# Autodesk Inventor assembly: EL2-GB-100
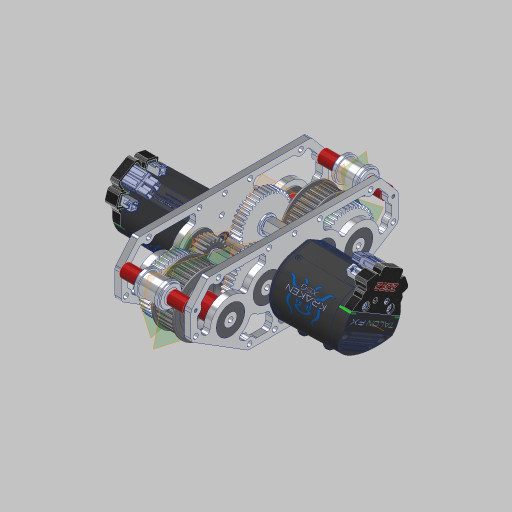
[picture p0: Inventor's stored thumbnail of the model, 512x512]
Saved by Autodesk Inventor 2023.5 (Build 275446000, 446)
## iProperties
Created: 2025-01-18
Part Number: EL2-GB-100
Document SubType Name: Assembly
Designer: jmcintyr
Author: jmcintyr
## Documents named in this file (17)
- C:\Users\slick\OneDrive\Desktop\2025-ReefScape---CAD\Elevator\EL2-GB\EL2-GB-100.iam
- C:\Users\slick\OneDrive\Desktop\2025-ReefScape---CAD\Elevator\EL2-GB\EL2-GB-001.ipt
- C:\Users\slick\OneDrive\Desktop\2025-ReefScape---CAD\Elevator\EL2-GB\EL2-GB-002.ipt
- C:\Users\slick\OneDrive\Desktop\2025-ReefScape---CAD\COMMON PARTS\MOTORS\Kracken with Cover and Boards.iam
- C:\Users\slick\OneDrive\Desktop\2025-ReefScape---CAD\COMMON PARTS\BEARINGS\0_500_ID_x_1_125_OD_x_0_313_WD_Flanged_Bearing_217-2731.ipt
- C:\Users\slick\OneDrive\Desktop\2025-ReefScape---CAD\COMMON PARTS\GEARS\20dp .5 hex\20t_Aluminum_Spur_Gear_20_DP_1_2_Hex_Bore_217-2702.ipt
- C:\Users\slick\OneDrive\Desktop\2025-ReefScape---CAD\COMMON PARTS\GEARS\20dp .5 hex\40t_Aluminum_Spur_Gear_20_DP_1_2_Hex_Bore_217-2708.ipt
- C:\Users\slick\OneDrive\Desktop\2025-ReefScape---CAD\COMMON PARTS\PULLEYS\htd\36t_x_15mm_Wide_Aluminum_Pulley_HTD_5mm_1_2_Hex_217-4103.ipt
- C:\Users\slick\OneDrive\Desktop\2025-ReefScape---CAD\Elevator\EL2-GB\EL2-GB-200.iam
- C:\Users\slick\OneDrive\Desktop\2025-ReefScape---CAD\Elevator\EL2-GB\EL2-GB-003.ipt
- C:\Users\slick\OneDrive\Desktop\2025-ReefScape---CAD\Elevator\EL2-GB\EL2-GB-004Spacer.ipt
- C:\Users\slick\OneDrive\Desktop\2025-ReefScape---CAD\Elevator\EL2-GB\EL2-GB-005E-grove.ipt
- C:\Users\slick\OneDrive\Desktop\2025-ReefScape---CAD\Elevator\EL2-GB\EL2-GB-006Spacer.ipt
- C:\Users\slick\OneDrive\Desktop\2025-ReefScape---CAD\Elevator\EL2-GB\EL2-GB-007Spacer.ipt
- C:\Users\slick\OneDrive\Desktop\2025-ReefScape---CAD\Elevator\EL2-GB\EL2-GB-008.ipt
- C:\Users\slick\OneDrive\Desktop\2025-ReefScape---CAD\Elevator\EL2-GB\EL2-GB-009Spacer.ipt
- C:\Users\slick\OneDrive\Desktop\2025-ReefScape---CAD\COMMON PARTS\GEARS\WCP-1006\WCP-1006.ipt
## Components (46 placed, 16 different names)
1. EL2-GB-001:1 — Insert:3, Insert:4, Insert:10, Insert:11, Insert:16, Insert:17, Insert:18, Insert:19, Symmetry:1, Mate:18, Mate:45, Insert:27, Mate:49
2. EL2-GB-001:2 — Insert:8, Insert:9, Insert:12, Insert:13, Insert:14, Insert:15, Symmetry:1, Insert:24, Insert:25, Insert:26, Mate:46, Mate:50
3. EL2-GB-002:1 — Insert:3, Insert:25
4. EL2-GB-002:5 — Insert:4, Insert:24
5. Kracken with Cover and Boards:1 [sub-assembly] — Insert:8, Insert:9
6. Kracken with Cover and Boards:2 [sub-assembly] — Insert:10, Insert:11
7. 0_500_ID_x_1_125_OD_x_0_313_WD_Flanged_Bearing_217-2731:1 — Insert:16, Mate:7, Insert:20, Mate:39, Mate:40
8. 0_500_ID_x_1_125_OD_x_0_313_WD_Flanged_Bearing_217-2731:2 — Insert:17, Insert:21, Mate:33, Mate:34, Mate:35
9. 0_500_ID_x_1_125_OD_x_0_313_WD_Flanged_Bearing_217-2731:3 — Insert:18, Mate:14
10. 0_500_ID_x_1_125_OD_x_0_313_WD_Flanged_Bearing_217-2731:4 — Insert:19, Mate:13, Insert:22, Mate:25, Mate:27
11. 0_500_ID_x_1_125_OD_x_0_313_WD_Flanged_Bearing_217-2731:5 — Insert:12, Mate:10, Mate:37, Mate:38, Mate:42
12. 0_500_ID_x_1_125_OD_x_0_313_WD_Flanged_Bearing_217-2731:6 — Insert:13, Mate:5, Mate:6, Mate:36
13. 0_500_ID_x_1_125_OD_x_0_313_WD_Flanged_Bearing_217-2731:7 — Insert:14, Mate:11, Insert:23, Mate:29, Mate:30, Mate:31
14. 0_500_ID_x_1_125_OD_x_0_313_WD_Flanged_Bearing_217-2731:8 — Insert:15, Mate:23
15. 20t_Aluminum_Spur_Gear_20_DP_1_2_Hex_Bore_217-2702:1 — Mate:6, Mate:22, Flush:4
16. 20t_Aluminum_Spur_Gear_20_DP_1_2_Hex_Bore_217-2702:2 — Mate:14, Mate:20, Flush:6, Mate:32
17. WCP-1006:1
18. WCP-1006:2
19. 40t_Aluminum_Spur_Gear_20_DP_1_2_Hex_Bore_217-2708:1 — Mate:11, Flush:5
20. 40t_Aluminum_Spur_Gear_20_DP_1_2_Hex_Bore_217-2708:2 — Mate:5
21. 40t_Aluminum_Spur_Gear_20_DP_1_2_Hex_Bore_217-2708:3 — Mate:7, Mate:22, Mate:41
22. 36t_x_15mm_Wide_Aluminum_Pulley_HTD_5mm_1_2_Hex_217-4103:1 — Mate:9, Mate:10, Mate:15
23. 40t_Aluminum_Spur_Gear_20_DP_1_2_Hex_Bore_217-2708:4 — Mate:13, Mate:16, Mate:20, Mate:28
24. 36t_x_15mm_Wide_Aluminum_Pulley_HTD_5mm_1_2_Hex_217-4103:2 — Mate:15, Mate:16, Mate:17, Mate:24, Mate:26
25. EL2-GB-200:1 [sub-assembly] — Mate:17, Mate:18
26. EL2-GB-005E-grove:2 — Insert:23, Flush:5, Flush:6
27. EL2-GB-003:2 — Insert:22
28. EL2-GB-005E-grove:1 — Insert:21, Flush:4
29. EL2-GB-003:4 — Insert:20
30. EL2-GB-004Spacer:1 — Mate:23, Mate:24
31. EL2-GB-006Spacer:1 — Mate:25, Mate:26
32. EL2-GB-007Spacer:1 — Mate:27, Mate:28
33. EL2-GB-007Spacer:2 — Mate:29, Mate:30
34. EL2-GB-007Spacer:3 — Mate:31, Mate:32
35. EL2-GB-007Spacer:4 — Mate:33, Mate:36
36. EL2-GB-007Spacer:5 — Mate:34, Mate:35
37. EL2-GB-007Spacer:6 — Mate:37, Mate:42
38. EL2-GB-006Spacer:2 — Mate:38, Mate:41
39. EL2-GB-004Spacer:2 — Mate:39, Mate:40
40. EL2-GB-008:1 — Insert:26, Mate:43, Mate:44
41. EL2-GB-009Spacer:1 — Mate:44, Mate:45
42. EL2-GB-009Spacer:2 — Mate:43, Mate:46
43. EL2-GB-200:2 [sub-assembly] — Flush:7, Mate:51
44. EL2-GB-008:2 — Insert:27, Mate:51
45. EL2-GB-009Spacer:3 — Mate:49
46. EL2-GB-009Spacer:4 — Mate:50
## Relationships (75: Mate 47, Insert 22, Flush 5, Symmetry 1)
- Insert:3: EL2-GB-001:1 ↔ EL2-GB-002:1
- Insert:4: EL2-GB-001:1 ↔ EL2-GB-002:5
- Insert:8: EL2-GB-001:2 ↔ Kracken with Cover and Boards:1
- Insert:9: EL2-GB-001:2 ↔ Kracken with Cover and Boards:1
- Insert:10: EL2-GB-001:1 ↔ Kracken with Cover and Boards:2
- Insert:11: EL2-GB-001:1 ↔ Kracken with Cover and Boards:2
- Insert:12: EL2-GB-001:2 ↔ 0_500_ID_x_1_125_OD_x_0_313_WD_Flanged_Bearing_217-2731:5
- Insert:13: EL2-GB-001:2 ↔ 0_500_ID_x_1_125_OD_x_0_313_WD_Flanged_Bearing_217-2731:6
- Insert:14: EL2-GB-001:2 ↔ 0_500_ID_x_1_125_OD_x_0_313_WD_Flanged_Bearing_217-2731:7
- Insert:15: EL2-GB-001:2 ↔ 0_500_ID_x_1_125_OD_x_0_313_WD_Flanged_Bearing_217-2731:8
- Insert:16: EL2-GB-001:1 ↔ 0_500_ID_x_1_125_OD_x_0_313_WD_Flanged_Bearing_217-2731:1
- Insert:17: EL2-GB-001:1 ↔ 0_500_ID_x_1_125_OD_x_0_313_WD_Flanged_Bearing_217-2731:2
- Insert:18: EL2-GB-001:1 ↔ 0_500_ID_x_1_125_OD_x_0_313_WD_Flanged_Bearing_217-2731:3
- Insert:19: EL2-GB-001:1 ↔ 0_500_ID_x_1_125_OD_x_0_313_WD_Flanged_Bearing_217-2731:4
- [Mate]: Kracken with Cover and Boards:1 ↔ WCP-1006:1
- [Mate]: Kracken with Cover and Boards:2 ↔ WCP-1006:2
- [Mate] (3.175 mm): EL2-GB-001:2 ↔ WCP-1006:1
- [Mate] (3.175 mm): EL2-GB-001:1 ↔ WCP-1006:2
- Mate:5: 0_500_ID_x_1_125_OD_x_0_313_WD_Flanged_Bearing_217-2731:6 ↔ 40t_Aluminum_Spur_Gear_20_DP_1_2_Hex_Bore_217-2708:2
- Mate:6: 0_500_ID_x_1_125_OD_x_0_313_WD_Flanged_Bearing_217-2731:6 ↔ 20t_Aluminum_Spur_Gear_20_DP_1_2_Hex_Bore_217-2702:1
- Mate:7: 0_500_ID_x_1_125_OD_x_0_313_WD_Flanged_Bearing_217-2731:1 ↔ 40t_Aluminum_Spur_Gear_20_DP_1_2_Hex_Bore_217-2708:3
- [Flush]: WCP-1006:2 ↔ 40t_Aluminum_Spur_Gear_20_DP_1_2_Hex_Bore_217-2708:2
- Symmetry:1: EL2-GB-001:1 ↔ EL2-GB-001:2
- Mate:9: 36t_x_15mm_Wide_Aluminum_Pulley_HTD_5mm_1_2_Hex_217-4103:1
- Mate:10: 0_500_ID_x_1_125_OD_x_0_313_WD_Flanged_Bearing_217-2731:5 ↔ 36t_x_15mm_Wide_Aluminum_Pulley_HTD_5mm_1_2_Hex_217-4103:1
- Mate:11: 0_500_ID_x_1_125_OD_x_0_313_WD_Flanged_Bearing_217-2731:7 ↔ 40t_Aluminum_Spur_Gear_20_DP_1_2_Hex_Bore_217-2708:1
- Mate:13: 0_500_ID_x_1_125_OD_x_0_313_WD_Flanged_Bearing_217-2731:4 ↔ 40t_Aluminum_Spur_Gear_20_DP_1_2_Hex_Bore_217-2708:4
- Mate:14: 0_500_ID_x_1_125_OD_x_0_313_WD_Flanged_Bearing_217-2731:3 ↔ 20t_Aluminum_Spur_Gear_20_DP_1_2_Hex_Bore_217-2702:2
- Mate:15: 36t_x_15mm_Wide_Aluminum_Pulley_HTD_5mm_1_2_Hex_217-4103:1 ↔ 36t_x_15mm_Wide_Aluminum_Pulley_HTD_5mm_1_2_Hex_217-4103:2
- Mate:16: 40t_Aluminum_Spur_Gear_20_DP_1_2_Hex_Bore_217-2708:4 ↔ 36t_x_15mm_Wide_Aluminum_Pulley_HTD_5mm_1_2_Hex_217-4103:2
- Mate:17: 36t_x_15mm_Wide_Aluminum_Pulley_HTD_5mm_1_2_Hex_217-4103:2 ↔ EL2-GB-200:1
- Mate:18: EL2-GB-001:1 ↔ EL2-GB-200:1
- Insert:20: 0_500_ID_x_1_125_OD_x_0_313_WD_Flanged_Bearing_217-2731:1 ↔ EL2-GB-003:4
- Insert:21: 0_500_ID_x_1_125_OD_x_0_313_WD_Flanged_Bearing_217-2731:2 ↔ EL2-GB-005E-grove:1
- Insert:22: 0_500_ID_x_1_125_OD_x_0_313_WD_Flanged_Bearing_217-2731:4 ↔ EL2-GB-003:2
- Insert:23: 0_500_ID_x_1_125_OD_x_0_313_WD_Flanged_Bearing_217-2731:7 ↔ EL2-GB-005E-grove:2
- Insert:24: EL2-GB-001:2 ↔ EL2-GB-002:5
- Insert:25: EL2-GB-001:2 ↔ EL2-GB-002:1
- Mate:20: 20t_Aluminum_Spur_Gear_20_DP_1_2_Hex_Bore_217-2702:2 ↔ 40t_Aluminum_Spur_Gear_20_DP_1_2_Hex_Bore_217-2708:4
- Mate:22: 20t_Aluminum_Spur_Gear_20_DP_1_2_Hex_Bore_217-2702:1 ↔ 40t_Aluminum_Spur_Gear_20_DP_1_2_Hex_Bore_217-2708:3
- Flush:4: 20t_Aluminum_Spur_Gear_20_DP_1_2_Hex_Bore_217-2702:1 ↔ EL2-GB-005E-grove:1
- Flush:5: 40t_Aluminum_Spur_Gear_20_DP_1_2_Hex_Bore_217-2708:1 ↔ EL2-GB-005E-grove:2
- Flush:6: 20t_Aluminum_Spur_Gear_20_DP_1_2_Hex_Bore_217-2702:2 ↔ EL2-GB-005E-grove:2
- Mate:23: 0_500_ID_x_1_125_OD_x_0_313_WD_Flanged_Bearing_217-2731:8 ↔ EL2-GB-004Spacer:1
- Mate:24: 36t_x_15mm_Wide_Aluminum_Pulley_HTD_5mm_1_2_Hex_217-4103:2 ↔ EL2-GB-004Spacer:1
- Mate:25: 0_500_ID_x_1_125_OD_x_0_313_WD_Flanged_Bearing_217-2731:4 ↔ EL2-GB-006Spacer:1
- Mate:26: 36t_x_15mm_Wide_Aluminum_Pulley_HTD_5mm_1_2_Hex_217-4103:2 ↔ EL2-GB-006Spacer:1
- Mate:27: 0_500_ID_x_1_125_OD_x_0_313_WD_Flanged_Bearing_217-2731:4 ↔ EL2-GB-007Spacer:1
- Mate:28: 40t_Aluminum_Spur_Gear_20_DP_1_2_Hex_Bore_217-2708:4 ↔ EL2-GB-007Spacer:1
- Mate:29: 0_500_ID_x_1_125_OD_x_0_313_WD_Flanged_Bearing_217-2731:7 ↔ EL2-GB-007Spacer:2
- Mate:30: 0_500_ID_x_1_125_OD_x_0_313_WD_Flanged_Bearing_217-2731:7 ↔ EL2-GB-007Spacer:2
- Mate:31: 0_500_ID_x_1_125_OD_x_0_313_WD_Flanged_Bearing_217-2731:7 ↔ EL2-GB-007Spacer:3
- Mate:32: 20t_Aluminum_Spur_Gear_20_DP_1_2_Hex_Bore_217-2702:2 ↔ EL2-GB-007Spacer:3
- Mate:33: 0_500_ID_x_1_125_OD_x_0_313_WD_Flanged_Bearing_217-2731:2 ↔ EL2-GB-007Spacer:4
- Mate:34: 0_500_ID_x_1_125_OD_x_0_313_WD_Flanged_Bearing_217-2731:2 ↔ EL2-GB-007Spacer:5
- Mate:35: 0_500_ID_x_1_125_OD_x_0_313_WD_Flanged_Bearing_217-2731:2 ↔ EL2-GB-007Spacer:5
- Mate:36: 0_500_ID_x_1_125_OD_x_0_313_WD_Flanged_Bearing_217-2731:6 ↔ EL2-GB-007Spacer:4
- Mate:37: 0_500_ID_x_1_125_OD_x_0_313_WD_Flanged_Bearing_217-2731:5 ↔ EL2-GB-007Spacer:6
- Mate:38: 0_500_ID_x_1_125_OD_x_0_313_WD_Flanged_Bearing_217-2731:5 ↔ EL2-GB-006Spacer:2
- Mate:39: 0_500_ID_x_1_125_OD_x_0_313_WD_Flanged_Bearing_217-2731:1 ↔ EL2-GB-004Spacer:2
- Mate:40: 0_500_ID_x_1_125_OD_x_0_313_WD_Flanged_Bearing_217-2731:1 ↔ EL2-GB-004Spacer:2
- Mate:41: 40t_Aluminum_Spur_Gear_20_DP_1_2_Hex_Bore_217-2708:3 ↔ EL2-GB-006Spacer:2
- Mate:42: 0_500_ID_x_1_125_OD_x_0_313_WD_Flanged_Bearing_217-2731:5 ↔ EL2-GB-007Spacer:6
- Insert:26: EL2-GB-001:2 ↔ EL2-GB-008:1
- Mate:43: EL2-GB-008:1 ↔ EL2-GB-009Spacer:2
- Mate:44: EL2-GB-008:1 ↔ EL2-GB-009Spacer:1
- Mate:45: EL2-GB-001:1 ↔ EL2-GB-009Spacer:1
- Mate:46: EL2-GB-001:2 ↔ EL2-GB-009Spacer:2
- [Mate]: EL2-GB-008:2 ↔ EL2-GB-009Spacer:4
- [Mate]: EL2-GB-008:2 ↔ EL2-GB-009Spacer:3
- Insert:27: EL2-GB-001:1 ↔ EL2-GB-008:2
- Mate:49: EL2-GB-001:1 ↔ EL2-GB-009Spacer:3
- Mate:50: EL2-GB-001:2 ↔ EL2-GB-009Spacer:4
- Flush:7: EL2-GB-200:2
- Mate:51: EL2-GB-200:2 ↔ EL2-GB-008:2
## Named parameters: d82_d78 = 0 mm, d83_d79 = 0 mm
